# Autodesk Inventor assembly: wrom gearbox nmrv 50
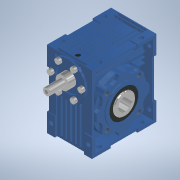
[picture p0: Inventor's stored thumbnail of the model, 180x180]
Saved by Autodesk Inventor 2020 (Build 240168000, 168)
## iProperties
Created: 2020-07-31
Part Number: wrom gearbox nmrv 50
Document SubType Name: Assembly
Designer: Vikki
Author: Vikki
## Documents named in this file (4)
- E:\project inventor pro\flipkart grid models\articulated arm\nmrv gear boxes\nmrv-50\wrom gearbox nmrv 50.iam
- E:\project inventor pro\flipkart grid models\articulated arm\nmrv 50 casing.ipt
- E:\project inventor pro\flipkart grid models\articulated arm\nmrv gear boxes\nmrv-50\inputshaft nmrv50.ipt
- E:\project inventor pro\flipkart grid models\articulated arm\nmrv gear boxes\nmrv-50\outputshaft nmrv50.ipt
## Components (3 placed, 3 different names)
1. nmrv 50 casing:1 — Mate:1, Mate:3, Flush:1, Mate:4
2. inputshaft nmrv50:1 — Mate:1, Rotation:1, Mate:4
3. outputshaft nmrv50:1 — Mate:3, Flush:1, Rotation:1
## Relationships (5: Mate 3, Flush 1, RelateRotation 1)
- Mate:1: nmrv 50 casing:1 ↔ inputshaft nmrv50:1
- Mate:3: nmrv 50 casing:1 ↔ outputshaft nmrv50:1
- Flush:1 (-1.5 mm): nmrv 50 casing:1 ↔ outputshaft nmrv50:1
- Rotation:1 [RelateRotation] (30 ul): inputshaft nmrv50:1 ↔ outputshaft nmrv50:1
- Mate:4: nmrv 50 casing:1 ↔ inputshaft nmrv50:1
